# Autodesk Inventor assembly: Ensamblaje completoo
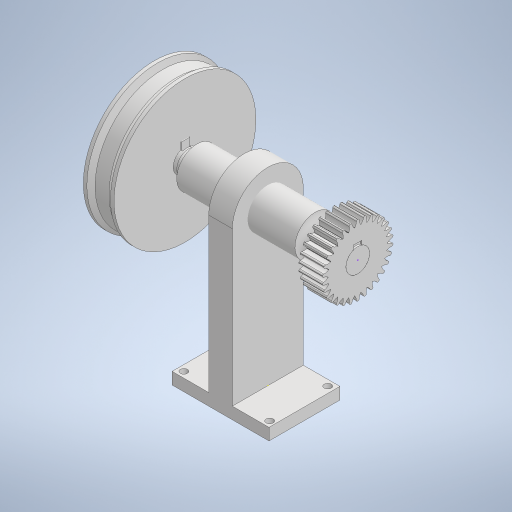
[picture p0: Inventor's stored thumbnail of the model, 512x512]
Saved by Autodesk Inventor 2024 (Build 280153000, 153)
## iProperties
Created: 2024-03-31
Part Number: Ensamblaje completoo
Document SubType Name: Assembly
Designer: Adrian Montalvan
Author: Adrian Montalvan
## Documents named in this file (6)
- C:\Users\Adrian Montalvan\Documents\ADRIAN\URL\11. 1er Semestre 2024\DINAMICA\A Dinamica Lab\Ensamble\Ensamblaje completoo.iam
- C:\Users\Adrian Montalvan\Documents\ADRIAN\URL\11. 1er Semestre 2024\DINAMICA\A Dinamica Lab\Ensamble\POLEA.ipt
- C:\Users\Adrian Montalvan\Documents\ADRIAN\URL\11. 1er Semestre 2024\DINAMICA\A Dinamica Lab\Ensamble\Pextra.ipt
- C:\Users\Adrian Montalvan\Documents\ADRIAN\URL\11. 1er Semestre 2024\DINAMICA\A Dinamica Lab\Ensamble\ENGRANE.ipt
- C:\Users\Adrian Montalvan\Documents\ADRIAN\URL\11. 1er Semestre 2024\DINAMICA\A Dinamica Lab\Ensamble\EJE_CUÑEROS.ipt
- C:\Users\Adrian Montalvan\Documents\ADRIAN\URL\11. 1er Semestre 2024\DINAMICA\A Dinamica Lab\Ensamble\CUÑA.ipt
## Components (6 placed, 5 different names)
1. POLEA:1 — De rotación:1
2. Pextra:1 — Rígido:3
3. ENGRANE:1 — De rotación:2
4. EJE_CUÑEROS:1 — Rígido:1, Rígido:2, De rotación:1, De rotación:2, Rígido:3
5. CUÑA:1 — Rígido:1
6. CUÑA:2 — Rígido:2
## Relationships (5: WeldJoint 3, RevoluteJoint 2)
- Rígido:1 [WeldJoint]: EJE_CUÑEROS:1 ↔ CUÑA:1
- Rígido:2 [WeldJoint]: EJE_CUÑEROS:1 ↔ CUÑA:2
- De rotación:1 [RevoluteJoint]: POLEA:1 ↔ EJE_CUÑEROS:1
- De rotación:2 [RevoluteJoint]: ENGRANE:1 ↔ EJE_CUÑEROS:1
- Rígido:3 [WeldJoint]: Pextra:1 ↔ EJE_CUÑEROS:1
